# Autodesk Inventor assembly: Assembly pesticide
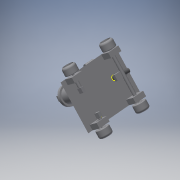
[picture p0: Inventor's stored thumbnail of the model, 180x180]
Saved by Autodesk Inventor 2019 (Build 230136000, 136)
## iProperties
Created: 2020-03-03
Part Number: Assembly pesticide
Document SubType Name: Assembly
Designer: dvg
Author: dvg
## Documents named in this file (16)
- C:\Users\dvg\Documents\Assembly pesticide.iam
- C:\Users\dvg\Documents\pesticide.ipt
- C:\Users\dvg\Documents\rod.ipt
- C:\Users\dvg\Documents\Part11.ipt
- C:\Users\dvg\Documents\tank lib 1.ipt
- C:\Users\dvg\Documents\Part13.ipt
- C:\Users\dvg\Documents\Wheels.ipt
- C:\Users\dvg\Documents\Part14.ipt
- C:\Users\dvg\Documents\Part17.ipt
- C:\Users\dvg\Documents\Part18.ipt
- C:\Users\dvg\Documents\Part19.ipt
- C:\Users\dvg\Documents\part21.ipt
- C:\Users\dvg\Documents\Part24.ipt
- C:\Users\dvg\Documents\Part25.ipt
- C:\Users\dvg\Documents\Part26.ipt
- C:\Users\dvg\Documents\Part28.ipt
## Components (23 placed, 15 different names)
1. pesticide:1 — Mate:1, Rotational:1, Slider:1, Rotational:2, Mate:2, Rotational:3, Mate:3, Slider:2, Rigid:1, Rotational:5, Rotational:6, Mate:4, Rotational:7, Mate:8, Mate:9, Mate:10
2. rod:1 — Mate:1, Rotational:1, Rotational:8, Rotational:9, Rotational:11, Rotational:14
3. Part11:1 — Slider:1, Mate:10, Rotational:10
4. tank lib 1:1 — Rotational:2
5. Part13:1 — Mate:2, Rotational:3, Mate:3, Slider:2, Slider:3, Rotational:4, Ball:1
6. Wheels:1 — Slider:3, Ball:1
7. Wheels:2 — Rotational:4
8. Wheels:3 — Rotational:5
9. Wheels:4 — Rigid:1
10. Part14:1 — Rotational:6
11. Part14:2 — Mate:4, Rotational:7
12. Part17:1 — Rotational:8, Mate:5, Mate:6, Mate:7
13. Part18:1 — Mate:5
14. Part19:1 — Mate:7
15. Part19:2 — Mate:6
16. part21:1 — Mate:8, Mate:9
17. Part24:2 — Rotational:9
18. Part25:1 — Rotational:10, Rotational:13
19. Part25:2 — Rotational:11, Rotational:12, Rotational:14
20. Part25:3 — Rotational:12, Mate:11
21. Part25:5 — Rotational:13, Mate:12, Rotational:15
22. Part26:1 — Mate:11, Mate:12
23. Part28:1 — Rotational:15
## Relationships (32: RevoluteJoint 15, Mate 12, TranslationJoint 3, WeldJoint 1, BallJoint 1)
- Mate:1: pesticide:1 ↔ rod:1
- Rotational:1 [RevoluteJoint]: pesticide:1 ↔ rod:1
- Slider:1 [TranslationJoint]: pesticide:1 ↔ Part11:1
- Rotational:2 [RevoluteJoint]: pesticide:1 ↔ tank lib 1:1
- Mate:2: pesticide:1 ↔ Part13:1
- Rotational:3 [RevoluteJoint]: pesticide:1 ↔ Part13:1
- Mate:3: pesticide:1 ↔ Part13:1
- Slider:2 [TranslationJoint]: pesticide:1 ↔ Part13:1
- Slider:3 [TranslationJoint] (2.54 mm): Part13:1 ↔ Wheels:1
- Rotational:4 [RevoluteJoint] (-2.54 mm): Part13:1 ↔ Wheels:2
- Rigid:1 [WeldJoint]: pesticide:1 ↔ Wheels:4
- Rotational:5 [RevoluteJoint]: pesticide:1 ↔ Wheels:3
- Rotational:6 [RevoluteJoint]: pesticide:1 ↔ Part14:1
- Mate:4: pesticide:1 ↔ Part14:2
- Rotational:7 [RevoluteJoint]: pesticide:1 ↔ Part14:2
- Ball:1: Part13:1 ↔ Wheels:1
- Rotational:8 [RevoluteJoint]: rod:1 ↔ Part17:1
- Mate:5: Part17:1 ↔ Part18:1
- Mate:6: Part17:1 ↔ Part19:2
- Mate:7: Part17:1 ↔ Part19:1
- Mate:8: pesticide:1 ↔ part21:1
- Mate:9: pesticide:1 ↔ part21:1
- Mate:10: pesticide:1 ↔ Part11:1
- Rotational:9 [RevoluteJoint]: rod:1 ↔ Part24:2
- Rotational:10 [RevoluteJoint]: Part11:1 ↔ Part25:1
- Rotational:11 [RevoluteJoint]: rod:1 ↔ Part25:2
- Rotational:12 [RevoluteJoint]: Part25:2 ↔ Part25:3
- Rotational:13 [RevoluteJoint]: Part25:1 ↔ Part25:5
- Rotational:14 [RevoluteJoint]: rod:1 ↔ Part25:2
- Mate:11: Part25:3 ↔ Part26:1
- Mate:12: Part25:5 ↔ Part26:1
- Rotational:15 [RevoluteJoint]: Part25:5 ↔ Part28:1
